# Autodesk Inventor assembly: 1x20Pins
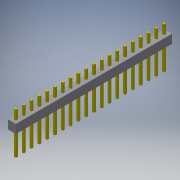
[picture p0: Inventor's stored thumbnail of the model, 180x180]
Saved by Autodesk Inventor 2019 (Build 230136000, 136)
## iProperties
Created: 2019-07-16
Part Number: 1x20Pins
Document SubType Name: Assembly
Designer: james
Author: james
## Documents named in this file (2)
- F:\JimsDesign\P1001-16bit-CPU\P1001-001 - 16bit CPU\P1001-001-210 - CAD Library\1x20Pins.iam
- F:\JimsDesign\P1001-16bit-CPU\P1001-001 - 16bit CPU\P1001-001-210 - CAD Library\1x4Pins.iam
## Components (5 placed, 1 different names)
1. 1x4Pins:1 [sub-assembly] — Mate:3, Mate:4, Flush:5, Flush:6, Flush:7, Flush:8
2. 1x4Pins:2 [sub-assembly] — Mate:4, Flush:6, Flush:8
3. 1x4Pins:3 [sub-assembly] — Mate:2, Flush:3, Flush:4, Mate:3, Flush:5, Flush:7
4. 1x4Pins:4 [sub-assembly] — Mate:1, Flush:1, Flush:2
5. 1x4Pins:5 [sub-assembly] — Mate:1, Mate:2, Flush:1, Flush:2, Flush:3, Flush:4
## Relationships (12: Flush 8, Mate 4)
- Mate:1: 1x4Pins:4 ↔ 1x4Pins:5
- Mate:2: 1x4Pins:3 ↔ 1x4Pins:5
- Flush:1: 1x4Pins:4 ↔ 1x4Pins:5
- Flush:2: 1x4Pins:4 ↔ 1x4Pins:5
- Flush:3: 1x4Pins:3 ↔ 1x4Pins:5
- Flush:4: 1x4Pins:3 ↔ 1x4Pins:5
- Mate:3: 1x4Pins:1 ↔ 1x4Pins:3
- Mate:4: 1x4Pins:1 ↔ 1x4Pins:2
- Flush:5: 1x4Pins:1 ↔ 1x4Pins:3
- Flush:6: 1x4Pins:1 ↔ 1x4Pins:2
- Flush:7: 1x4Pins:1 ↔ 1x4Pins:3
- Flush:8: 1x4Pins:1 ↔ 1x4Pins:2
